# Autodesk Inventor assembly: CC-module
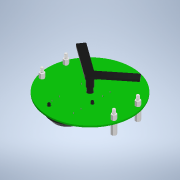
[picture p0: Inventor's stored thumbnail of the model, 180x180]
Saved by Autodesk Inventor 2020 (Build 240168000, 168)
## iProperties
Created: 2019-07-03
Part Number: CC-module
Document SubType Name: Assembly
Designer: andwh
Author: andwh
## Documents named in this file (7)
- C:\Users\andwh\Documents\Projects\Clock Clock\CC-module.iam
- C:\Users\andwh\Documents\Projects\Clock Clock\CC-PCB.ipt
- C:\Users\andwh\Documents\Projects\Clock Clock\Parts\BKA30D-R5.ipt
- C:\Users\andwh\Documents\Projects\Clock Clock\Parts\95783A051_NYLON 6-6 MALE-FEM THRDED HEX STANDOFF.ipt
- C:\Users\andwh\Documents\Projects\Clock Clock\Parts\95783A059_NYLON 6-6 MALE-FEM THRDED HEX STANDOFF.ipt
- C:\Users\andwh\Documents\Projects\Clock Clock\CC-bottomHand.ipt
- C:\Users\andwh\Documents\Projects\Clock Clock\CC-topHand.ipt
## Components (12 placed, 6 different names)
1. CC-PCB:1 — Insert:1, Insert:2, Insert:3, Insert:4
2. BKA30D-R5:1 — Insert:1, Insert:2, Insert:5, Insert:6
3. CC-bottomHand:1 — Insert:5
4. CC-topHand:1 — Insert:6
5. 95783A051_NYLON 6-6 MALE-FEM THRDED HEX STANDOFF:1 — Insert:3
6. 95783A059_NYLON 6-6 MALE-FEM THRDED HEX STANDOFF:1 — Insert:4
7. 95783A051_NYLON 6-6 MALE-FEM THRDED HEX STANDOFF:2
8. 95783A059_NYLON 6-6 MALE-FEM THRDED HEX STANDOFF:2
9. 95783A051_NYLON 6-6 MALE-FEM THRDED HEX STANDOFF:3
10. 95783A059_NYLON 6-6 MALE-FEM THRDED HEX STANDOFF:3
11. 95783A051_NYLON 6-6 MALE-FEM THRDED HEX STANDOFF:4
12. 95783A059_NYLON 6-6 MALE-FEM THRDED HEX STANDOFF:4
## Component patterns: (4 elements, first: 95783A051_NYLON 6-6 MALE-FEM THRDED HEX STANDOFF:1 + 95783A059_NYLON 6-6 MALE-FEM THRDED HEX STANDOFF:1)
## Relationships (6: Insert 6)
- Insert:1: CC-PCB:1 ↔ BKA30D-R5:1
- Insert:2: CC-PCB:1 ↔ BKA30D-R5:1
- Insert:3: CC-PCB:1 ↔ 95783A051_NYLON 6-6 MALE-FEM THRDED HEX STANDOFF:1
- Insert:4: CC-PCB:1 ↔ 95783A059_NYLON 6-6 MALE-FEM THRDED HEX STANDOFF:1
- Insert:5: BKA30D-R5:1 ↔ CC-bottomHand:1
- Insert:6: BKA30D-R5:1 ↔ CC-topHand:1
